# Autodesk Inventor assembly: Assembly1
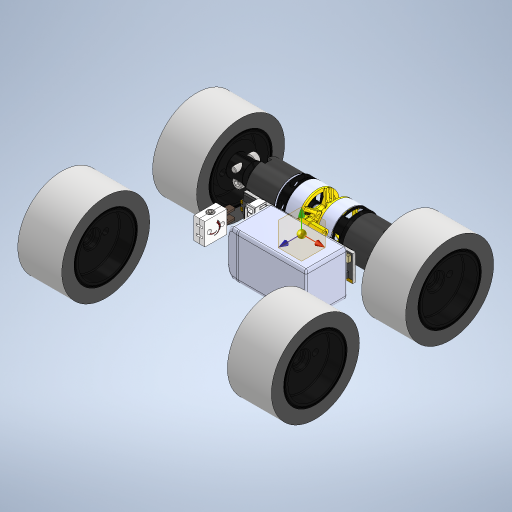
[picture p0: Inventor's stored thumbnail of the model, 512x512]
Saved by Autodesk Inventor 2023.2 (Build 272271000, 271)
## iProperties
Created: 2023-01-11
Part Number: Assembly1
Document SubType Name: Assembly
Designer: Nathan Cai
Mass: 331.27 g
Surface Area: 778.778 cm^2
Volume: 164.727 cm^3
Density: 2.01102 g/cm^3
Author: Nathan Cai
## Documents named in this file (7)
- E:\Documents\Inventor\IMchass V3.0\Drive Pod 1.iam
- E:\Documents\Inventor\IMchass V3.0\RR Brushless\RR-Brushless-Planetary.iam
- E:\Documents\Inventor\IMchass V3.0\D2_Narrow_Wheels_2.75in_x_1in.ipt
- E:\Documents\Inventor\IMchass V3.0\Botkit-Hubs.ipt
- E:\Documents\Inventor\IMchass V3.0\Tattu 4S 850mah\Tattu 850mah 4S.iam
- E:\Documents\Inventor\IMchass V3.0\RDQ ESC32.ipt
- E:\Documents\Inventor\IMchass V3.0\Fingertech Power Switch\Fingertech Mini Power Switch.iam
## Components (12 placed, 6 different names)
1. RR-Brushless-Planetary:1 [sub-assembly] — Mate:1, Mate:2, Mate:5
2. D2_Narrow_Wheels_2.75in_x_1in:1 — Mate:7
3. D2_Narrow_Wheels_2.75in_x_1in:2 — Mate:6
4. Botkit-Hubs:1 — Mate:1, Mate:2
5. RR-Brushless-Planetary:2 [sub-assembly] — Mate:5
6. Botkit-Hubs:2
7. D2_Narrow_Wheels_2.75in_x_1in:3 — Mate:7
8. D2_Narrow_Wheels_2.75in_x_1in:4 — Mate:6
9. Tattu 850mah 4S:1 [sub-assembly]
10. RDQ ESC32:1
11. RDQ ESC32:2
12. Fingertech Mini Power Switch:1 [sub-assembly]
## Relationships (7: Mate 7)
- Mate:1: RR-Brushless-Planetary:1 ↔ Botkit-Hubs:1
- Mate:2: RR-Brushless-Planetary:1 ↔ Botkit-Hubs:1
- [Mate]: RR-Brushless-Planetary:2 ↔ Botkit-Hubs:2
- [Mate]: RR-Brushless-Planetary:2 ↔ Botkit-Hubs:2
- Mate:5: RR-Brushless-Planetary:1 ↔ RR-Brushless-Planetary:2
- Mate:6: D2_Narrow_Wheels_2.75in_x_1in:2 ↔ D2_Narrow_Wheels_2.75in_x_1in:4
- Mate:7: D2_Narrow_Wheels_2.75in_x_1in:1 ↔ D2_Narrow_Wheels_2.75in_x_1in:3
## Named parameters: d2_d0 = 0 mm, d3_d1 = 0 mm
